# Autodesk Inventor assembly: Filament Path Components
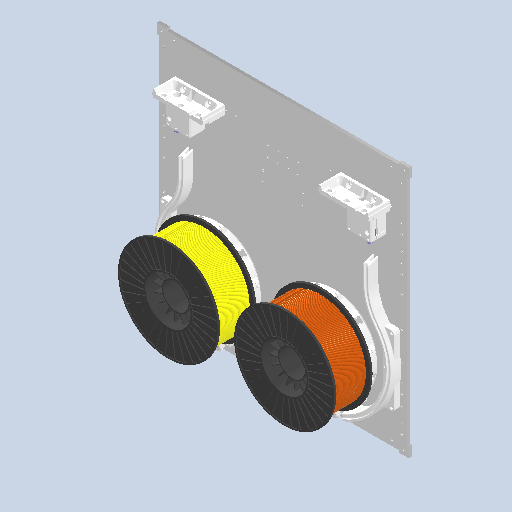
[picture p0: Inventor's stored thumbnail of the model, 512x512]
Saved by Autodesk Inventor 2024 (Build 280153000, 153)
## iProperties
Created: 2024-08-19
Part Number: Filament Path Components
Document SubType Name: Assembly
Designer: Ishaan
Author: Ishaan
## Documents named in this file (10)
- E:\Projects\Axiom--IDEX-3D-Printer\CAD\05 - Filament Path\Filament Path Components.iam
- E:\Projects\Axiom--IDEX-3D-Printer\CAD\02 - Frame\Printer Base Plate RevI.ipt
- E:\Projects\Axiom--IDEX-3D-Printer\CAD\05 - Filament Path\Filament Motion Sensor Left.iam
- E:\Projects\Axiom--IDEX-3D-Printer\CAD\05 - Filament Path\Filament Motion Sensor Right.iam
- E:\Projects\Axiom--IDEX-3D-Printer\CAD\05 - Filament Path\Spool Holder Assembly.iam
- E:\Projects\Axiom--IDEX-3D-Printer\CAD\05 - Filament Path\Sample Filament Spool 2.ipt
- E:\Projects\Axiom--IDEX-3D-Printer\CAD\05 - Filament Path\Sample Filament Spool.ipt
- E:\Projects\Axiom--IDEX-3D-Printer\CAD\05 - Filament Path\Filament Inlet Guide Left.ipt
- E:\Projects\Axiom--IDEX-3D-Printer\CAD\00 - COTS Components\16mm LED Pushbutton\16mm LED Pushbutton.ipt
- E:\Projects\Axiom--IDEX-3D-Printer\CAD\05 - Filament Path\Filament Inlet Guide Right.ipt
## Components (11 placed, 9 different names)
1. Printer Base Plate RevI:1 — Insert:1, Insert:2, Insert:3, Insert:4, Insert:5, Insert:6, Insert:7, Insert:8, Insert:9, Insert:10, Insert:11, Insert:12, Insert:13, Insert:14, Insert:15, Insert:16, Insert:17, Insert:18, Insert:19, Insert:20, Insert:22, Insert:23, Insert:24, Insert:25
2. Filament Motion Sensor Left:1 [sub-assembly] — Insert:1, Insert:2
3. Filament Motion Sensor Right:1 [sub-assembly] — Insert:3, Insert:4
4. Spool Holder Assembly:1 [sub-assembly] — Insert:5, Insert:6, Insert:7, Insert:8, Insert:9, Insert:10, Mate:1, Mate:2
5. Spool Holder Assembly:2 [sub-assembly] — Insert:11, Insert:12, Insert:13, Insert:14, Insert:15, Insert:16, Mate:3, Mate:4
6. Sample Filament Spool 2:1 — Mate:1, Mate:2
7. Sample Filament Spool:1 — Mate:3, Mate:4
8. Filament Inlet Guide Left:1 — Insert:17, Insert:18, Insert:19, Insert:20, Insert:21
9. 16mm LED Pushbutton:1 — Insert:21
10. Filament Inlet Guide Right:1 — Insert:22, Insert:23, Insert:24, Insert:25, Insert:26
11. 16mm LED Pushbutton:2 — Insert:26
## Relationships (30: Insert 26, Mate 4)
- Insert:1: Printer Base Plate RevI:1 ↔ Filament Motion Sensor Left:1
- Insert:2: Printer Base Plate RevI:1 ↔ Filament Motion Sensor Left:1
- Insert:3: Printer Base Plate RevI:1 ↔ Filament Motion Sensor Right:1
- Insert:4: Printer Base Plate RevI:1 ↔ Filament Motion Sensor Right:1
- Insert:5: Printer Base Plate RevI:1 ↔ Spool Holder Assembly:1
- Insert:6: Printer Base Plate RevI:1 ↔ Spool Holder Assembly:1
- Insert:7: Printer Base Plate RevI:1 ↔ Spool Holder Assembly:1
- Insert:8: Printer Base Plate RevI:1 ↔ Spool Holder Assembly:1
- Insert:9: Printer Base Plate RevI:1 ↔ Spool Holder Assembly:1
- Insert:10: Printer Base Plate RevI:1 ↔ Spool Holder Assembly:1
- Insert:11: Printer Base Plate RevI:1 ↔ Spool Holder Assembly:2
- Insert:12: Printer Base Plate RevI:1 ↔ Spool Holder Assembly:2
- Insert:13: Printer Base Plate RevI:1 ↔ Spool Holder Assembly:2
- Insert:14: Printer Base Plate RevI:1 ↔ Spool Holder Assembly:2
- Insert:15: Printer Base Plate RevI:1 ↔ Spool Holder Assembly:2
- Insert:16: Printer Base Plate RevI:1 ↔ Spool Holder Assembly:2
- Mate:1: Spool Holder Assembly:1 ↔ Sample Filament Spool 2:1
- Mate:2: Spool Holder Assembly:1 ↔ Sample Filament Spool 2:1
- Mate:3: Spool Holder Assembly:2 ↔ Sample Filament Spool:1
- Mate:4: Spool Holder Assembly:2 ↔ Sample Filament Spool:1
- Insert:17: Printer Base Plate RevI:1 ↔ Filament Inlet Guide Left:1
- Insert:18: Printer Base Plate RevI:1 ↔ Filament Inlet Guide Left:1
- Insert:19: Printer Base Plate RevI:1 ↔ Filament Inlet Guide Left:1
- Insert:20: Printer Base Plate RevI:1 ↔ Filament Inlet Guide Left:1
- Insert:21: Filament Inlet Guide Left:1 ↔ 16mm LED Pushbutton:1
- Insert:22: Printer Base Plate RevI:1 ↔ Filament Inlet Guide Right:1
- Insert:23: Printer Base Plate RevI:1 ↔ Filament Inlet Guide Right:1
- Insert:24: Printer Base Plate RevI:1 ↔ Filament Inlet Guide Right:1
- Insert:25: Printer Base Plate RevI:1 ↔ Filament Inlet Guide Right:1
- Insert:26: Filament Inlet Guide Right:1 ↔ 16mm LED Pushbutton:2
